# Autodesk Inventor assembly: Two stage cylindrical spur gear reducer with lateral offset
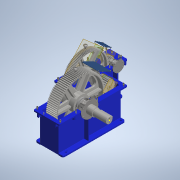
[picture p0: Inventor's stored thumbnail of the model, 180x180]
Saved by Autodesk Inventor 2020 (Build 240168000, 168)
## iProperties
Part Number: Two stage cylindrical spur gear reducer with lateral offset
Document SubType Name: 部件
Designer: chenpeizhi66
Author: PeiZhi Chen
## Documents named in this file (59)
- C:\Users\dell\Desktop\最终上交\爆炸图\装配3\Workspace\cpz assemble.iam
- C:\Users\dell\Desktop\最终上交\爆炸图\装配3\Libraries\Content Center Files\zh-CN\GB_T 283 (NUP)\滚动轴承 NUP NUP 208 E GB_T 283.ipt
- C:\Users\dell\Desktop\最终上交\爆炸图\装配3\Libraries\Content Center Files\zh-CN\GB_T 283 (NUP)\滚动轴承 NUP NUP 2313 E GB_T 283.ipt
- C:\Users\dell\Desktop\最终上交\爆炸图\装配3\Libraries\Content Center Files\zh-CN\GB_T 276-94\滚动轴承 61922 GB_T 276-94.ipt
- C:\Users\dell\Desktop\最终上交\爆炸图\装配3\Workspace\xia(1).ipt
- C:\Users\dell\Desktop\最终上交\爆炸图\装配3\Workspace\轴1.ipt
- C:\Users\dell\Desktop\最终上交\爆炸图\装配3\Workspace\轴2.ipt
- C:\Users\dell\Desktop\最终上交\爆炸图\装配3\Workspace\轴3.ipt
- C:\Users\dell\Desktop\最终上交\爆炸图\装配3\Workspace\挡油板2.ipt
- C:\Users\dell\Desktop\最终上交\爆炸图\装配3\Workspace\轴套1.ipt
- C:\Users\dell\Desktop\最终上交\爆炸图\装配3\Workspace\key1.ipt
- C:\Users\dell\Desktop\最终上交\爆炸图\装配3\Workspace\key2.ipt
- C:\Users\dell\Desktop\最终上交\爆炸图\装配3\Workspace\key3.ipt
- C:\Users\dell\Desktop\最终上交\爆炸图\装配3\Workspace\key5.ipt
- C:\Users\dell\Desktop\最终上交\爆炸图\装配3\Workspace\shaft_try_1\设计加速器\正齿轮11.ipt
- C:\Users\dell\Desktop\最终上交\爆炸图\装配3\Workspace\shaft_try_1\设计加速器\正齿轮12.ipt
- C:\Users\dell\Desktop\最终上交\爆炸图\装配3\Workspace\shaft_try_1\设计加速器\正齿轮21.ipt
- C:\Users\dell\Desktop\最终上交\爆炸图\装配3\Workspace\shaft_try_1\设计加速器\正齿轮22.ipt
- C:\Users\dell\Desktop\最终上交\爆炸图\装配3\Workspace\轴套3.ipt
- C:\Users\dell\Desktop\最终上交\爆炸图\装配3\Workspace\轴端挡圈.ipt
- C:\Users\dell\Desktop\最终上交\爆炸图\装配3\Workspace\螺栓 GB 32.1 M6 x 30.ipt
- C:\Users\dell\Desktop\最终上交\爆炸图\装配3\Workspace\轴套2.ipt
- C:\Users\dell\Desktop\最终上交\爆炸图\装配3\Workspace\弹性挡圈GB 894.1-86 - 40.ipt
- C:\Users\dell\Desktop\最终上交\爆炸图\装配3\Workspace\弹性挡圈GB 894.1-86 - 70.ipt
- C:\Users\dell\Desktop\最终上交\爆炸图\装配3\Workspace\轴4.ipt
- C:\Users\dell\Desktop\最终上交\爆炸图\装配3\Workspace\油塞1.ipt
- C:\Users\dell\Desktop\最终上交\爆炸图\装配3\Workspace\shang(1).ipt
- C:\Users\dell\Desktop\最终上交\爆炸图\装配3\Libraries\Content Center Files\zh-CN\GB_T 6175-2000\螺母 GB_T 6175 M10.ipt
- C:\Users\dell\Desktop\最终上交\爆炸图\装配3\Workspace\螺栓 GB_T 5785 M12 x 1.5 x 110.ipt
- C:\Users\dell\Desktop\最终上交\爆炸图\装配3\Workspace\螺栓 GB_T 5785 M12 x 1.5 x 45.ipt
- C:\Users\dell\Desktop\最终上交\爆炸图\装配3\Libraries\Content Center Files\zh-CN\GB 93-87\垫圈 GB 93-87 12.ipt
- C:\Users\dell\Desktop\最终上交\爆炸图\装配3\Workspace\螺母 GB_T 6175 M10.ipt
- C:\Users\dell\Desktop\最终上交\爆炸图\装配3\Workspace\视空盖1.ipt
- C:\Users\dell\Desktop\最终上交\爆炸图\装配3\Workspace\视孔盖2.ipt
- C:\Users\dell\Desktop\最终上交\爆炸图\装配3\Workspace\通气器1.ipt
- C:\Users\dell\Desktop\最终上交\爆炸图\装配3\Workspace\螺栓 GB_T 5783 M6 x 14.ipt
- C:\Users\dell\Desktop\最终上交\爆炸图\装配3\Libraries\Content Center Files\zh-CN\GB_T 5783-2000\螺栓 GB_T 5783 M6 x 14.ipt
- C:\Users\dell\Desktop\最终上交\爆炸图\装配3\Workspace\垫片1.ipt
- C:\Users\dell\Desktop\最终上交\爆炸图\装配3\Workspace\轴承端盖1.ipt
- C:\Users\dell\Desktop\最终上交\爆炸图\装配3\Workspace\O 形密封圈  P- 37.5 x 2.65-G-GB_T 3452.1-2005.ipt
- C:\Users\dell\Desktop\最终上交\爆炸图\装配3\Workspace\轴承端盖2.ipt
- C:\Users\dell\Desktop\最终上交\爆炸图\装配3\Workspace\垫片2.ipt
- C:\Users\dell\Desktop\最终上交\爆炸图\装配3\Workspace\垫片3.ipt
- C:\Users\dell\Desktop\最终上交\爆炸图\装配3\Workspace\垫片4.ipt
- C:\Users\dell\Desktop\最终上交\爆炸图\装配3\Workspace\轴承盖挡圈.ipt
- C:\Users\dell\Desktop\最终上交\爆炸图\装配3\Workspace\轴承通盖1.ipt
- C:\Users\dell\Desktop\最终上交\爆炸图\装配3\Workspace\轴承端盖3.ipt
- C:\Users\dell\Desktop\最终上交\爆炸图\装配3\Workspace\轴承通盖.ipt
- C:\Users\dell\Desktop\最终上交\爆炸图\装配3\Workspace\螺母 GB 810 M30 x 1.5.ipt
- C:\Users\dell\Desktop\最终上交\爆炸图\装配3\Libraries\Content Center Files\zh-CN\GB 858-88\垫圈 GB 858 30.ipt
- C:\Users\dell\Desktop\最终上交\爆炸图\装配3\Workspace\垫圈 GB 858 64.ipt
- C:\Users\dell\Desktop\最终上交\爆炸图\装配3\Workspace\螺母 GB 810 M64 x 2.ipt
- C:\Users\dell\Desktop\最终上交\爆炸图\装配3\Workspace\油塞垫.ipt
- C:\Users\dell\Desktop\最终上交\爆炸图\装配3\Workspace\锥形销 GB_T 117 A 10 x 40.ipt
- C:\Users\dell\Desktop\最终上交\爆炸图\装配3\Libraries\Content Center Files\zh-CN\GB_T 5782-2000\螺栓 GB_T 5782 M10 x 35.ipt
- C:\Users\dell\Desktop\最终上交\爆炸图\装配3\Workspace\零件2.ipt
- C:\Users\dell\Desktop\最终上交\爆炸图\装配3\Libraries\Content Center Files\zh-CN\GB 831-88\螺钉 GB 831 M8 x 6.ipt
- C:\Users\dell\Desktop\最终上交\爆炸图\装配3\Workspace\零件1.ipt
- C:\Users\dell\Desktop\最终上交\爆炸图\装配3\Workspace\零件3.ipt
## Components (146 placed, 54 different names)
1. 滚动轴承 GB/T 283 NUP 型 NUP 208 E:1 — 配合:2, 配合:18, 配合:54
2. 滚动轴承 GB/T 283 NUP 型 NUP 2313 E:1 — 配合:13, 配合:50, 配合:52
3. 滚动轴承 GB/T 283 NUP 型 NUP 208 E:2 — 配合:4, 配合:6, 配合:8, 配合:330, 配合:331, 配合:338
4. 滚动轴承 GB/T 283 NUP 型 NUP 2313 E:2 — 配合:14, 配合:15, 配合:16, 配合:334
5. 滚动轴承 GB/T 276-1994 60000 和 160000 型 61922:1 — 配合:23, 配合:29, 配合:419
6. 滚动轴承 GB/T 276-1994 60000 和 160000 型 61922:2 — 配合:24, 配合:38, 配合:418
7. xia(1):1 — 配合:2, 配合:4, 总驱动, 配合:5, 配合:11, 配合:12, 配合:13, 配合:14, 配合:15, 配合:23, 配合:24, 配合:59, 配合:60, 配合:65, 表面齐平:1, 表面齐平:2, 配合:66, 配合:67, 配合:68, 配合:69, 配合:70, 配合:71, 配合:72, 配合:73, 配合:74, 配合:75, 配合:76, 配合:77, 配合:78, 配合:79, 配合:80, 配合:81, 配合:82, 配合:83, 配合:84, 配合:85, 配合:108, 配合:109, 配合:110, 配合:111, 配合:112, 配合:113, 配合:114, 配合:115, 配合:116, 配合:117, 配合:118, 配合:119, 表面齐平:3, 表面齐平:4, 表面齐平:5, 表面齐平:6, 配合:298, 配合:307, 角度:2, 配合:318, 配合:319, 配合:320, 配合:322, 角度:3, 配合:327, 配合:340, 配合:341, 配合:342, 配合:344, 配合:345, 配合:346, 配合:362, 配合:364, 配合:366, 配合:368, 配合:370, 配合:372, 配合:374, 配合:376, 配合:388, 配合:390, 配合:392, 配合:400, 配合:402, 配合:404, 配合:416
8. shang(1):1 — 配合:65, 表面齐平:1, 表面齐平:2, 配合:163, 配合:165, 配合:167, 配合:169, 配合:171, 配合:173, 配合:175, 配合:177, 配合:179, 配合:181, 配合:183, 配合:185, 配合:187, 配合:189, 配合:191, 配合:193, 表面齐平:3, 表面齐平:4, 表面齐平:5, 表面齐平:6, 配合:269, 配合:270, 配合:271, 配合:272, 配合:273, 配合:274, 配合:275, 配合:276, 配合:277, 配合:278, 配合:279, 配合:281, 配合:283, 配合:285, 配合:287, 配合:289, 配合:291, 配合:293, 配合:299, 配合:308, 配合:312, 配合:314, 配合:315, 配合:349, 配合:350, 配合:352, 配合:354, 配合:356, 配合:358, 配合:360, 配合:378, 配合:380, 配合:382, 配合:384, 配合:386, 配合:394, 配合:396, 配合:398, 配合:407, 配合:408, 配合:409, 配合:410, 配合:411, 配合:412, 配合:413, 配合:414, 配合:415, 配合:417
9. 轴:1 — 配合:11, 刚性:3, 转动:1, 配合:16, 刚性:8, 配合:19, 配合:20, 转动:2, 配合:46, 配合:47, 配合:48, 配合:51, 配合:306, 配合:309, 配合:333, 配合:335, 刚性:10
10. 轴:2 — 配合:12, 转动:2, 配合:22, 配合:29, 配合:36, 配合:311, 配合:313, 配合:324, 配合:326, 刚性:11, 刚性:12
11. 驱动轴 — 总驱动, 配合:5, 配合:6, 配合:7, 配合:9, 刚性:1, 刚性:2, 配合:10, 转动:1, 配合:53, 配合:297, 配合:304, 配合:329, 配合:337
12. 挡油板2:1 — 配合:7, 配合:8, 配合:9
13. 轴套1:1 — 配合:10, 配合:17, 配合:18
14. key1:1 — 刚性:1
15. key2:1 — 刚性:2, 刚性:7
16. key3:1 — 刚性:3
17. key5:1 — 刚性:12, 配合:420
18. 正齿轮1:2 — 刚性:7, 配合:17
19. 正齿轮2:1 — 配合:22, 配合:37, 配合:420
20. 正齿轮2:2 — 刚性:8, 配合:49
21. 轴套3:1 — 配合:36, 配合:37, 配合:38
22. 轴端挡圈:1 — 配合:41, 配合:42, 配合:43, 配合:44, 配合:45, 对称:1
23. 螺栓 GB 32.1 M6 x 30:1 — 配合:43, 配合:45, 配合:47
24. 螺栓 GB 32.1 M6 x 30:2 — 配合:42, 配合:44, 配合:46, 对称:1, 表面齐平:9
25. 轴套2:1 — 配合:48, 配合:49, 配合:50
26. 弹性挡圈GB 894.1-86 - 40:1 — 配合:53, 配合:54
27. 弹性挡圈GB 894.1-86 - 70:1 — 配合:51, 配合:52
28. 轴:4 — 配合:59, 配合:60
29. 螺栓 GB_T 5785 M12 x 1.5 x 110:1 — 配合:66, 配合:67, 配合:132, 配合:164
30. 螺栓 GB_T 5785 M12 x 1.5 x 110:2 — 配合:68, 配合:69, 配合:178, 配合:208
31. 螺栓 GB_T 5785 M12 x 1.5 x 110:3 — 配合:70, 配合:71, 配合:136, 配合:168
32. 螺栓 GB_T 5785 M12 x 1.5 x 110:4 — 配合:72, 配合:73, 配合:186, 配合:216
33. 螺栓 GB_T 5785 M12 x 1.5 x 110:5 — 配合:74, 配合:75, 配合:134, 配合:166
34. 螺栓 GB_T 5785 M12 x 1.5 x 110:6 — 配合:76, 配合:77, 配合:106, 配合:162
35. 螺栓 GB_T 5785 M12 x 1.5 x 110:7 — 配合:78, 配合:79, 配合:184, 配合:214
36. 螺栓 GB_T 5785 M12 x 1.5 x 110:8 — 配合:80, 配合:81, 配合:188, 配合:218
37. 螺栓 GB_T 5785 M12 x 1.5 x 110:9 — 配合:82, 配合:83, 配合:180, 配合:210
38. 螺栓 GB_T 5785 M12 x 1.5 x 110:10 — 配合:84, 配合:85, 配合:172, 配合:202
39. 螺母 GB_T 6175 M10:1 — 配合:106, 配合:195
40. 螺栓 GB_T 5785 M12 x 1.5 x 45:1 — 配合:108, 配合:109, 配合:176, 配合:206
41. 螺栓 GB_T 5785 M12 x 1.5 x 45:2 — 配合:110, 配合:111, 配合:174, 配合:204
42. 螺栓 GB_T 5785 M12 x 1.5 x 45:3 — 配合:112, 配合:113, 配合:182, 配合:212
43. 螺栓 GB_T 5785 M12 x 1.5 x 45:4 — 配合:114, 配合:115, 配合:192, 配合:200
44. 螺栓 GB_T 5785 M12 x 1.5 x 45:5 — 配合:116, 配合:117, 配合:190, 配合:220
45. 螺栓 GB_T 5785 M12 x 1.5 x 45:6 — 配合:118, 配合:119, 配合:138, 配合:170
46. 螺母 GB_T 6175 M10:2 — 配合:132, 配合:196
47. 螺母 GB_T 6175 M10:3 — 配合:134, 配合:197
48. 螺母 GB_T 6175 M10:4 — 配合:136, 配合:198
49. 螺母 GB_T 6175 M10:5 — 配合:138, 配合:199
50. 垫圈 GB/T 93-1987 M12:1 — 配合:162, 配合:163, 配合:195
51. 垫圈 GB/T 93-1987 M12:2 — 配合:164, 配合:165, 配合:196
52. 垫圈 GB/T 93-1987 M12:3 — 配合:166, 配合:167, 配合:197
53. 垫圈 GB/T 93-1987 M12:4 — 配合:168, 配合:169, 配合:198
54. 垫圈 GB/T 93-1987 M12:5 — 配合:170, 配合:171, 配合:199
55. 垫圈 GB/T 93-1987 M12:6 — 配合:172, 配合:173, 配合:203
56. 垫圈 GB/T 93-1987 M12:7 — 配合:174, 配合:175, 配合:205
57. 垫圈 GB/T 93-1987 M12:8 — 配合:176, 配合:177, 配合:207
58. 垫圈 GB/T 93-1987 M12:9 — 配合:178, 配合:179, 配合:209
59. 垫圈 GB/T 93-1987 M12:10 — 配合:180, 配合:181, 配合:211
60. 垫圈 GB/T 93-1987 M12:11 — 配合:182, 配合:183, 配合:213
61. 垫圈 GB/T 93-1987 M12:12 — 配合:184, 配合:185, 配合:215
62. 垫圈 GB/T 93-1987 M12:13 — 配合:186, 配合:187, 配合:217
63. 垫圈 GB/T 93-1987 M12:14 — 配合:188, 配合:189, 配合:219
64. 垫圈 GB/T 93-1987 M12:15 — 配合:190, 配合:191, 配合:221
65. 垫圈 GB/T 93-1987 M12:16 — 配合:192, 配合:193, 配合:201
66. 螺母 GB/T 6175-2000 M10:1 — 配合:200, 配合:201
67. 螺母 GB/T 6175-2000 M10:2 — 配合:202, 配合:203
68. 螺母 GB/T 6175-2000 M10:3 — 配合:204, 配合:205
69. 螺母 GB/T 6175-2000 M10:4 — 配合:206, 配合:207
70. 螺母 GB/T 6175-2000 M10:5 — 配合:208, 配合:209
71. 螺母 GB/T 6175-2000 M10:6 — 配合:210, 配合:211
72. 螺母 GB/T 6175-2000 M10:7 — 配合:212, 配合:213
73. 螺母 GB/T 6175-2000 M10:8 — 配合:214, 配合:215
74. 螺母 GB/T 6175-2000 M10:9 — 配合:216, 配合:217
75. 螺母 GB/T 6175-2000 M10:10 — 配合:218, 配合:219
76. 螺母 GB/T 6175-2000 M10:11 — 配合:220, 配合:221
77. 视空盖1:1 — 配合:273, 配合:274, 配合:278, 配合:280, 配合:282, 配合:284, 配合:286
78. 视孔盖2:1 — 配合:275, 配合:276, 配合:277, 配合:288, 配合:290, 配合:292, 配合:294
79. 通气器1:1 — 配合:271, 配合:272
80. 通气器1:2 — 配合:269, 配合:270
81. 螺栓 GB_T 5783 M6 x 14:1 — 配合:279, 配合:280
82. 螺栓 GB_T 5783 M6 x 14:2 — 配合:281, 配合:282
83. 螺栓 GB_T 5783 M6 x 14:3 — 配合:283, 配合:284
84. 螺栓 GB_T 5783 M6 x 14:4 — 配合:285, 配合:286
85. 螺栓 GB/T 5783-2000 M6 x 14:1 — 配合:287, 配合:288
86. 螺栓 GB/T 5783-2000 M6 x 14:2 — 配合:289, 配合:290
87. 螺栓 GB/T 5783-2000 M6 x 14:3 — 配合:291, 配合:292
88. 螺栓 GB/T 5783-2000 M6 x 14:4 — 配合:293, 配合:294
89. 垫片1:1 — 配合:297, 配合:298, 配合:299, 配合:305
90. 轴承端盖1:1 — 配合:301, 配合:302, 配合:303, 配合:304, 配合:305, 配合:351, 配合:353, 配合:355, 配合:357, 配合:359, 配合:361, 配合:363, 配合:365, 配合:367, 配合:369, 配合:371, 配合:373
91. O 形密封圈  P- 37.5 x 2.65-G-GB_T 3452.1-2005:1 — 配合:301, 配合:302, 配合:303
92. 轴承端盖2:1 — 配合:309, 配合:310
93. 垫片2:1 — 配合:306, 配合:307, 配合:308, 配合:310
94. 垫片3:1 — 配合:311, 角度:2, 配合:312, 配合:325
95. 垫片4:1 — 配合:313, 配合:314, 配合:315, 配合:328
96. 垫片1:2 — 配合:318, 配合:319, 配合:320, 配合:323
97. 轴承通盖1:1 — 配合:322, 配合:323, 配合:395, 配合:397, 配合:399, 配合:401, 配合:403, 配合:405
98. 轴承端盖3:1 — 配合:324, 角度:3, 配合:325, 配合:375, 配合:377, 配合:379, 配合:381, 配合:419
99. 轴承通盖:1 — 配合:326, 配合:327, 配合:328, 配合:383, 配合:385, 配合:387, 配合:389, 配合:391, 配合:393, 配合:418, 表面齐平:7
100. 螺母 GB 810 M30 x 1.5:1 — 配合:331, 配合:332
101. 垫圈 GB/T 858-1988 30 x 40:1 — 配合:329, 配合:330, 配合:332
102. 垫圈 GB 858 64:1 — 配合:333, 配合:334, 配合:336
103. 螺母 GB 810 M64 x 2:1 — 配合:335, 配合:336
104. 轴承盖挡圈:2 — 配合:337, 配合:338
105. 油塞1:2 — 配合:342, 配合:343
106. 油塞垫:1 — 配合:344, 配合:345, 配合:347
107. 油塞垫:2 — 配合:340, 配合:341, 配合:343
108. 油塞1:3 — 配合:346, 配合:347
109. 锥形销 GB_T 117 A 10 x 40:1 — 配合:349, 配合:416
110. 螺栓 GB/T 5782-2000 M10x35:1 — 配合:350, 配合:351
111. 螺栓 GB/T 5782-2000 M10x35:2 — 配合:352, 配合:353
112. 螺栓 GB/T 5782-2000 M10x35:3 — 配合:354, 配合:355
113. 螺栓 GB/T 5782-2000 M10x35:4 — 配合:356, 配合:357
114. 螺栓 GB/T 5782-2000 M10x35:5 — 配合:358, 配合:359
115. 螺栓 GB/T 5782-2000 M10x35:6 — 配合:360, 配合:361
116. 螺栓 GB/T 5782-2000 M10x35:7 — 配合:362, 配合:363
117. 螺栓 GB/T 5782-2000 M10x35:8 — 配合:364, 配合:365
118. 螺栓 GB/T 5782-2000 M10x35:9 — 配合:366, 配合:367
119. 螺栓 GB/T 5782-2000 M10x35:10 — 配合:368, 配合:369
120. 螺栓 GB/T 5782-2000 M10x35:11 — 配合:370, 配合:371
121. 螺栓 GB/T 5782-2000 M10x35:12 — 配合:372, 配合:373
122. 螺栓 GB/T 5782-2000 M10x35:13 — 配合:374, 配合:375
123. 螺栓 GB/T 5782-2000 M10x35:14 — 配合:376, 配合:377
124. 螺栓 GB/T 5782-2000 M10x35:15 — 配合:378, 配合:379
125. 螺栓 GB/T 5782-2000 M10x35:16 — 配合:380, 配合:381
126. 螺栓 GB/T 5782-2000 M10x35:17 — 配合:382, 配合:383
127. 螺栓 GB/T 5782-2000 M10x35:18 — 配合:384, 配合:385
128. 螺栓 GB/T 5782-2000 M10x35:19 — 配合:386, 配合:387
129. 螺栓 GB/T 5782-2000 M10x35:20 — 配合:388, 配合:389
130. 螺栓 GB/T 5782-2000 M10x35:21 — 配合:390, 配合:391
131. 螺栓 GB/T 5782-2000 M10x35:22 — 配合:392, 配合:393
132. 螺栓 GB/T 5782-2000 M10x35:23 — 配合:394, 配合:395
133. 螺栓 GB/T 5782-2000 M10x35:24 — 配合:396, 配合:397
134. 螺栓 GB/T 5782-2000 M10x35:25 — 配合:398, 配合:399
135. 螺栓 GB/T 5782-2000 M10x35:26 — 配合:400, 配合:401
136. 螺栓 GB/T 5782-2000 M10x35:27 — 配合:402, 配合:403
137. 螺栓 GB/T 5782-2000 M10x35:28 — 配合:404, 配合:405
138. 零件2:1 — 刚性:10, 配合:406
139. 螺钉 GB/T 831-1988 M8 x 6:1 — 配合:407, 配合:408
140. 螺钉 GB/T 831-1988 M8 x 6:2 — 配合:409, 配合:417
141. 螺钉 GB/T 831-1988 M8 x 6:3 — 配合:410, 配合:414
142. 螺钉 GB/T 831-1988 M8 x 6:4 — 配合:411, 配合:413
143. 螺钉 GB/T 831-1988 M8 x 6:5 — 配合:412, 配合:415
144. 零件1:1 — 刚性:11
145. 零件3:1 — 表面齐平:7, 表面齐平:8, 表面齐平:9
146. 正齿轮1:1 — 配合:19, 配合:20, 配合:41, 配合:406
## Relationships (305: Mate 282, Flush 9, WeldJoint 8, Angle 3, RelateRotation 2, Symmetry 1)
- 配合:2 [Mate]: 滚动轴承 GB/T 283 NUP 型 NUP 208 E:1 ↔ xia(1):1
- 配合:4 [Mate]: 滚动轴承 GB/T 283 NUP 型 NUP 208 E:2 ↔ xia(1):1
- 总驱动 [Angle] (104 deg): xia(1):1 ↔ 驱动轴
- 配合:5 [Mate]: xia(1):1 ↔ 驱动轴
- 配合:6 [Mate]: 滚动轴承 GB/T 283 NUP 型 NUP 208 E:2 ↔ 驱动轴
- 配合:7 [Mate]: 驱动轴 ↔ 挡油板2:1
- 配合:8 [Mate]: 滚动轴承 GB/T 283 NUP 型 NUP 208 E:2 ↔ 挡油板2:1
- 配合:9 [Mate]: 驱动轴 ↔ 挡油板2:1
- 刚性:1 [WeldJoint]: 驱动轴 ↔ key1:1
- 刚性:2 [WeldJoint]: 驱动轴 ↔ key2:1
- 配合:10 [Mate]: 驱动轴 ↔ 轴套1:1
- 配合:11 [Mate]: xia(1):1 ↔ 轴:1
- 配合:12 [Mate]: xia(1):1 ↔ 轴:2
- 刚性:3 [WeldJoint]: 轴:1 ↔ key3:1
- 刚性:7 [WeldJoint]: key2:1 ↔ 正齿轮1:2
- 转动:1 [RelateRotation] (0.615 ul): 轴:1 ↔ 驱动轴
- 配合:13 [Mate]: 滚动轴承 GB/T 283 NUP 型 NUP 2313 E:1 ↔ xia(1):1
- 配合:14 [Mate]: 滚动轴承 GB/T 283 NUP 型 NUP 2313 E:2 ↔ xia(1):1
- 配合:15 [Mate]: 滚动轴承 GB/T 283 NUP 型 NUP 2313 E:2 ↔ xia(1):1
- 配合:16 [Mate]: 滚动轴承 GB/T 283 NUP 型 NUP 2313 E:2 ↔ 轴:1
- 配合:17 [Mate]: 轴套1:1 ↔ 正齿轮1:2
- 配合:18 [Mate]: 滚动轴承 GB/T 283 NUP 型 NUP 208 E:1 ↔ 轴套1:1
- 刚性:8 [WeldJoint]: 轴:1 ↔ 正齿轮2:2
- 配合:19 [Mate]: 轴:1 ↔ 正齿轮1:1
- 配合:20 [Mate]: 轴:1 ↔ 正齿轮1:1
- 转动:2 [RelateRotation] (1.833 ul): 轴:1 ↔ 轴:2
- 配合:22 [Mate]: 轴:2 ↔ 正齿轮2:1
- 配合:23 [Mate]: 滚动轴承 GB/T 276-1994 60000 和 160000 型 61922:1 ↔ xia(1):1
- 配合:24 [Mate]: 滚动轴承 GB/T 276-1994 60000 和 160000 型 61922:2 ↔ xia(1):1
- 配合:29 [Mate]: 滚动轴承 GB/T 276-1994 60000 和 160000 型 61922:1 ↔ 轴:2
- 配合:36 [Mate]: 轴:2 ↔ 轴套3:1
- 配合:37 [Mate]: 正齿轮2:1 ↔ 轴套3:1
- 配合:38 [Mate]: 滚动轴承 GB/T 276-1994 60000 和 160000 型 61922:2 ↔ 轴套3:1
- 配合:41 [Mate]: 轴端挡圈:1 ↔ 正齿轮1:1
- 配合:42 [Mate]: 轴端挡圈:1 ↔ 螺栓 GB 32.1 M6 x 30:2
- 配合:43 [Mate]: 轴端挡圈:1 ↔ 螺栓 GB 32.1 M6 x 30:1
- 配合:44 [Mate]: 轴端挡圈:1 ↔ 螺栓 GB 32.1 M6 x 30:2
- 配合:45 [Mate]: 轴端挡圈:1 ↔ 螺栓 GB 32.1 M6 x 30:1
- 配合:46 [Mate]: 轴:1 ↔ 螺栓 GB 32.1 M6 x 30:2
- 配合:47 [Mate]: 轴:1 ↔ 螺栓 GB 32.1 M6 x 30:1
- 配合:48 [Mate]: 轴:1 ↔ 轴套2:1
- 配合:49 [Mate]: 正齿轮2:2 ↔ 轴套2:1
- 配合:50 [Mate]: 滚动轴承 GB/T 283 NUP 型 NUP 2313 E:1 ↔ 轴套2:1
- 配合:51 [Mate]: 轴:1 ↔ 弹性挡圈GB 894.1-86 - 70:1
- 配合:52 [Mate]: 滚动轴承 GB/T 283 NUP 型 NUP 2313 E:1 ↔ 弹性挡圈GB 894.1-86 - 70:1
- 配合:53 [Mate]: 驱动轴 ↔ 弹性挡圈GB 894.1-86 - 40:1
- 配合:54 [Mate]: 滚动轴承 GB/T 283 NUP 型 NUP 208 E:1 ↔ 弹性挡圈GB 894.1-86 - 40:1
- 配合:59 [Mate]: xia(1):1 ↔ 轴:4
- 配合:60 [Mate]: xia(1):1 ↔ 轴:4
- 配合:65 [Mate]: xia(1):1 ↔ shang(1):1
- 表面齐平:1 [Flush]: xia(1):1 ↔ shang(1):1
- 表面齐平:2 [Flush]: xia(1):1 ↔ shang(1):1
- 配合:66 [Mate]: xia(1):1 ↔ 螺栓 GB_T 5785 M12 x 1.5 x 110:1
- 配合:67 [Mate]: xia(1):1 ↔ 螺栓 GB_T 5785 M12 x 1.5 x 110:1
- 配合:68 [Mate]: xia(1):1 ↔ 螺栓 GB_T 5785 M12 x 1.5 x 110:2
- 配合:69 [Mate]: xia(1):1 ↔ 螺栓 GB_T 5785 M12 x 1.5 x 110:2
- 配合:70 [Mate]: xia(1):1 ↔ 螺栓 GB_T 5785 M12 x 1.5 x 110:3
- 配合:71 [Mate]: xia(1):1 ↔ 螺栓 GB_T 5785 M12 x 1.5 x 110:3
- 配合:72 [Mate]: xia(1):1 ↔ 螺栓 GB_T 5785 M12 x 1.5 x 110:4
- 配合:73 [Mate]: xia(1):1 ↔ 螺栓 GB_T 5785 M12 x 1.5 x 110:4
- 配合:74 [Mate]: xia(1):1 ↔ 螺栓 GB_T 5785 M12 x 1.5 x 110:5
- 配合:75 [Mate]: xia(1):1 ↔ 螺栓 GB_T 5785 M12 x 1.5 x 110:5
- 配合:76 [Mate]: xia(1):1 ↔ 螺栓 GB_T 5785 M12 x 1.5 x 110:6
- 配合:77 [Mate]: xia(1):1 ↔ 螺栓 GB_T 5785 M12 x 1.5 x 110:6
- 配合:78 [Mate]: xia(1):1 ↔ 螺栓 GB_T 5785 M12 x 1.5 x 110:7
- 配合:79 [Mate]: xia(1):1 ↔ 螺栓 GB_T 5785 M12 x 1.5 x 110:7
- 配合:80 [Mate]: xia(1):1 ↔ 螺栓 GB_T 5785 M12 x 1.5 x 110:8
- 配合:81 [Mate]: xia(1):1 ↔ 螺栓 GB_T 5785 M12 x 1.5 x 110:8
- 配合:82 [Mate]: xia(1):1 ↔ 螺栓 GB_T 5785 M12 x 1.5 x 110:9
- 配合:83 [Mate]: xia(1):1 ↔ 螺栓 GB_T 5785 M12 x 1.5 x 110:9
- 配合:84 [Mate]: xia(1):1 ↔ 螺栓 GB_T 5785 M12 x 1.5 x 110:10
- 配合:85 [Mate]: xia(1):1 ↔ 螺栓 GB_T 5785 M12 x 1.5 x 110:10
- 配合:106 [Mate]: 螺栓 GB_T 5785 M12 x 1.5 x 110:6 ↔ 螺母 GB_T 6175 M10:1
- 配合:108 [Mate]: xia(1):1 ↔ 螺栓 GB_T 5785 M12 x 1.5 x 45:1
- 配合:109 [Mate]: xia(1):1 ↔ 螺栓 GB_T 5785 M12 x 1.5 x 45:1
- 配合:110 [Mate]: xia(1):1 ↔ 螺栓 GB_T 5785 M12 x 1.5 x 45:2
- 配合:111 [Mate]: xia(1):1 ↔ 螺栓 GB_T 5785 M12 x 1.5 x 45:2
- 配合:112 [Mate]: xia(1):1 ↔ 螺栓 GB_T 5785 M12 x 1.5 x 45:3
- 配合:113 [Mate]: xia(1):1 ↔ 螺栓 GB_T 5785 M12 x 1.5 x 45:3
- 配合:114 [Mate]: xia(1):1 ↔ 螺栓 GB_T 5785 M12 x 1.5 x 45:4
- 配合:115 [Mate]: xia(1):1 ↔ 螺栓 GB_T 5785 M12 x 1.5 x 45:4
- 配合:116 [Mate]: xia(1):1 ↔ 螺栓 GB_T 5785 M12 x 1.5 x 45:5
- 配合:117 [Mate]: xia(1):1 ↔ 螺栓 GB_T 5785 M12 x 1.5 x 45:5
- 配合:118 [Mate]: xia(1):1 ↔ 螺栓 GB_T 5785 M12 x 1.5 x 45:6
- 配合:119 [Mate]: xia(1):1 ↔ 螺栓 GB_T 5785 M12 x 1.5 x 45:6
- 配合:132 [Mate]: 螺栓 GB_T 5785 M12 x 1.5 x 110:1 ↔ 螺母 GB_T 6175 M10:2
- 配合:134 [Mate]: 螺栓 GB_T 5785 M12 x 1.5 x 110:5 ↔ 螺母 GB_T 6175 M10:3
- 配合:136 [Mate]: 螺栓 GB_T 5785 M12 x 1.5 x 110:3 ↔ 螺母 GB_T 6175 M10:4
- 配合:138 [Mate]: 螺栓 GB_T 5785 M12 x 1.5 x 45:6 ↔ 螺母 GB_T 6175 M10:5
- 配合:162 [Mate]: 螺栓 GB_T 5785 M12 x 1.5 x 110:6 ↔ 垫圈 GB/T 93-1987 M12:1
- 配合:163 [Mate]: shang(1):1 ↔ 垫圈 GB/T 93-1987 M12:1
- 配合:164 [Mate]: 螺栓 GB_T 5785 M12 x 1.5 x 110:1 ↔ 垫圈 GB/T 93-1987 M12:2
- 配合:165 [Mate]: shang(1):1 ↔ 垫圈 GB/T 93-1987 M12:2
- 配合:166 [Mate]: 螺栓 GB_T 5785 M12 x 1.5 x 110:5 ↔ 垫圈 GB/T 93-1987 M12:3
- 配合:167 [Mate]: shang(1):1 ↔ 垫圈 GB/T 93-1987 M12:3
- 配合:168 [Mate]: 螺栓 GB_T 5785 M12 x 1.5 x 110:3 ↔ 垫圈 GB/T 93-1987 M12:4
- 配合:169 [Mate]: shang(1):1 ↔ 垫圈 GB/T 93-1987 M12:4
- 配合:170 [Mate]: 螺栓 GB_T 5785 M12 x 1.5 x 45:6 ↔ 垫圈 GB/T 93-1987 M12:5
- 配合:171 [Mate]: shang(1):1 ↔ 垫圈 GB/T 93-1987 M12:5
- 配合:172 [Mate]: 螺栓 GB_T 5785 M12 x 1.5 x 110:10 ↔ 垫圈 GB/T 93-1987 M12:6
- 配合:173 [Mate]: shang(1):1 ↔ 垫圈 GB/T 93-1987 M12:6
- 配合:174 [Mate]: 螺栓 GB_T 5785 M12 x 1.5 x 45:2 ↔ 垫圈 GB/T 93-1987 M12:7
- 配合:175 [Mate]: shang(1):1 ↔ 垫圈 GB/T 93-1987 M12:7
- 配合:176 [Mate]: 螺栓 GB_T 5785 M12 x 1.5 x 45:1 ↔ 垫圈 GB/T 93-1987 M12:8
- 配合:177 [Mate]: shang(1):1 ↔ 垫圈 GB/T 93-1987 M12:8
- 配合:178 [Mate]: 螺栓 GB_T 5785 M12 x 1.5 x 110:2 ↔ 垫圈 GB/T 93-1987 M12:9
- 配合:179 [Mate]: shang(1):1 ↔ 垫圈 GB/T 93-1987 M12:9
- 配合:180 [Mate]: 螺栓 GB_T 5785 M12 x 1.5 x 110:9 ↔ 垫圈 GB/T 93-1987 M12:10
- 配合:181 [Mate]: shang(1):1 ↔ 垫圈 GB/T 93-1987 M12:10
- 配合:182 [Mate]: 螺栓 GB_T 5785 M12 x 1.5 x 45:3 ↔ 垫圈 GB/T 93-1987 M12:11
- 配合:183 [Mate]: shang(1):1 ↔ 垫圈 GB/T 93-1987 M12:11
- 配合:184 [Mate]: 螺栓 GB_T 5785 M12 x 1.5 x 110:7 ↔ 垫圈 GB/T 93-1987 M12:12
- 配合:185 [Mate]: shang(1):1 ↔ 垫圈 GB/T 93-1987 M12:12
- 配合:186 [Mate]: 螺栓 GB_T 5785 M12 x 1.5 x 110:4 ↔ 垫圈 GB/T 93-1987 M12:13
- 配合:187 [Mate]: shang(1):1 ↔ 垫圈 GB/T 93-1987 M12:13
- 配合:188 [Mate]: 螺栓 GB_T 5785 M12 x 1.5 x 110:8 ↔ 垫圈 GB/T 93-1987 M12:14
- 配合:189 [Mate]: shang(1):1 ↔ 垫圈 GB/T 93-1987 M12:14
- 配合:190 [Mate]: 螺栓 GB_T 5785 M12 x 1.5 x 45:5 ↔ 垫圈 GB/T 93-1987 M12:15
- 配合:191 [Mate]: shang(1):1 ↔ 垫圈 GB/T 93-1987 M12:15
- 配合:192 [Mate]: 螺栓 GB_T 5785 M12 x 1.5 x 45:4 ↔ 垫圈 GB/T 93-1987 M12:16
- 配合:193 [Mate]: shang(1):1 ↔ 垫圈 GB/T 93-1987 M12:16
- 配合:195 [Mate]: 螺母 GB_T 6175 M10:1 ↔ 垫圈 GB/T 93-1987 M12:1
- 配合:196 [Mate]: 螺母 GB_T 6175 M10:2 ↔ 垫圈 GB/T 93-1987 M12:2
- 配合:197 [Mate]: 螺母 GB_T 6175 M10:3 ↔ 垫圈 GB/T 93-1987 M12:3
- 配合:198 [Mate]: 螺母 GB_T 6175 M10:4 ↔ 垫圈 GB/T 93-1987 M12:4
- 配合:199 [Mate]: 螺母 GB_T 6175 M10:5 ↔ 垫圈 GB/T 93-1987 M12:5
- 配合:200 [Mate]: 螺栓 GB_T 5785 M12 x 1.5 x 45:4 ↔ 螺母 GB/T 6175-2000 M10:1
- 配合:201 [Mate]: 垫圈 GB/T 93-1987 M12:16 ↔ 螺母 GB/T 6175-2000 M10:1
- 配合:202 [Mate]: 螺栓 GB_T 5785 M12 x 1.5 x 110:10 ↔ 螺母 GB/T 6175-2000 M10:2
- 配合:203 [Mate]: 垫圈 GB/T 93-1987 M12:6 ↔ 螺母 GB/T 6175-2000 M10:2
- 配合:204 [Mate]: 螺栓 GB_T 5785 M12 x 1.5 x 45:2 ↔ 螺母 GB/T 6175-2000 M10:3
- 配合:205 [Mate]: 垫圈 GB/T 93-1987 M12:7 ↔ 螺母 GB/T 6175-2000 M10:3
- 配合:206 [Mate]: 螺栓 GB_T 5785 M12 x 1.5 x 45:1 ↔ 螺母 GB/T 6175-2000 M10:4
- 配合:207 [Mate]: 垫圈 GB/T 93-1987 M12:8 ↔ 螺母 GB/T 6175-2000 M10:4
- 配合:208 [Mate]: 螺栓 GB_T 5785 M12 x 1.5 x 110:2 ↔ 螺母 GB/T 6175-2000 M10:5
- 配合:209 [Mate]: 垫圈 GB/T 93-1987 M12:9 ↔ 螺母 GB/T 6175-2000 M10:5
- 配合:210 [Mate]: 螺栓 GB_T 5785 M12 x 1.5 x 110:9 ↔ 螺母 GB/T 6175-2000 M10:6
- 配合:211 [Mate]: 垫圈 GB/T 93-1987 M12:10 ↔ 螺母 GB/T 6175-2000 M10:6
- 配合:212 [Mate]: 螺栓 GB_T 5785 M12 x 1.5 x 45:3 ↔ 螺母 GB/T 6175-2000 M10:7
- 配合:213 [Mate]: 垫圈 GB/T 93-1987 M12:11 ↔ 螺母 GB/T 6175-2000 M10:7
- 配合:214 [Mate]: 螺栓 GB_T 5785 M12 x 1.5 x 110:7 ↔ 螺母 GB/T 6175-2000 M10:8
- 配合:215 [Mate]: 垫圈 GB/T 93-1987 M12:12 ↔ 螺母 GB/T 6175-2000 M10:8
- 配合:216 [Mate]: 螺栓 GB_T 5785 M12 x 1.5 x 110:4 ↔ 螺母 GB/T 6175-2000 M10:9
- 配合:217 [Mate]: 垫圈 GB/T 93-1987 M12:13 ↔ 螺母 GB/T 6175-2000 M10:9
- 配合:218 [Mate]: 螺栓 GB_T 5785 M12 x 1.5 x 110:8 ↔ 螺母 GB/T 6175-2000 M10:10
- 配合:219 [Mate]: 垫圈 GB/T 93-1987 M12:14 ↔ 螺母 GB/T 6175-2000 M10:10
- 配合:220 [Mate]: 螺栓 GB_T 5785 M12 x 1.5 x 45:5 ↔ 螺母 GB/T 6175-2000 M10:11
- 配合:221 [Mate]: 垫圈 GB/T 93-1987 M12:15 ↔ 螺母 GB/T 6175-2000 M10:11
- 表面齐平:3 [Flush]: xia(1):1 ↔ shang(1):1
- 表面齐平:4 [Flush]: xia(1):1 ↔ shang(1):1
- 表面齐平:5 [Flush]: xia(1):1 ↔ shang(1):1
- 表面齐平:6 [Flush]: xia(1):1 ↔ shang(1):1
- 配合:269 [Mate]: shang(1):1 ↔ 通气器1:2
- 配合:270 [Mate]: shang(1):1 ↔ 通气器1:2
- 配合:271 [Mate]: shang(1):1 ↔ 通气器1:1
- 配合:272 [Mate]: shang(1):1 ↔ 通气器1:1
- 配合:273 [Mate]: shang(1):1 ↔ 视空盖1:1
- 配合:274 [Mate]: shang(1):1 ↔ 视空盖1:1
- 配合:275 [Mate]: shang(1):1 ↔ 视孔盖2:1
- 配合:276 [Mate]: shang(1):1 ↔ 视孔盖2:1
- 配合:277 [Mate]: shang(1):1 ↔ 视孔盖2:1
- 配合:278 [Mate]: shang(1):1 ↔ 视空盖1:1
- 配合:279 [Mate]: shang(1):1 ↔ 螺栓 GB_T 5783 M6 x 14:1
- 配合:280 [Mate]: 视空盖1:1 ↔ 螺栓 GB_T 5783 M6 x 14:1
- 配合:281 [Mate]: shang(1):1 ↔ 螺栓 GB_T 5783 M6 x 14:2
- 配合:282 [Mate]: 视空盖1:1 ↔ 螺栓 GB_T 5783 M6 x 14:2
- 配合:283 [Mate]: shang(1):1 ↔ 螺栓 GB_T 5783 M6 x 14:3
- 配合:284 [Mate]: 视空盖1:1 ↔ 螺栓 GB_T 5783 M6 x 14:3
- 配合:285 [Mate]: shang(1):1 ↔ 螺栓 GB_T 5783 M6 x 14:4
- 配合:286 [Mate]: 视空盖1:1 ↔ 螺栓 GB_T 5783 M6 x 14:4
- 配合:287 [Mate]: shang(1):1 ↔ 螺栓 GB/T 5783-2000 M6 x 14:1
- 配合:288 [Mate]: 视孔盖2:1 ↔ 螺栓 GB/T 5783-2000 M6 x 14:1
- 配合:289 [Mate]: shang(1):1 ↔ 螺栓 GB/T 5783-2000 M6 x 14:2
- 配合:290 [Mate]: 视孔盖2:1 ↔ 螺栓 GB/T 5783-2000 M6 x 14:2
- 配合:291 [Mate]: shang(1):1 ↔ 螺栓 GB/T 5783-2000 M6 x 14:3
- 配合:292 [Mate]: 视孔盖2:1 ↔ 螺栓 GB/T 5783-2000 M6 x 14:3
- 配合:293 [Mate]: shang(1):1 ↔ 螺栓 GB/T 5783-2000 M6 x 14:4
- 配合:294 [Mate]: 视孔盖2:1 ↔ 螺栓 GB/T 5783-2000 M6 x 14:4
- 配合:297 [Mate]: 驱动轴 ↔ 垫片1:1
- 配合:298 [Mate]: xia(1):1 ↔ 垫片1:1
- 配合:299 [Mate]: shang(1):1 ↔ 垫片1:1
- 配合:301 [Mate]: 轴承端盖1:1 ↔ O 形密封圈  P- 37.5 x 2.65-G-GB_T 3452.1-2005:1
- 配合:302 [Mate]: 轴承端盖1:1 ↔ O 形密封圈  P- 37.5 x 2.65-G-GB_T 3452.1-2005:1
- 配合:303 [Mate]: 轴承端盖1:1 ↔ O 形密封圈  P- 37.5 x 2.65-G-GB_T 3452.1-2005:1
- 配合:304 [Mate]: 驱动轴 ↔ 轴承端盖1:1
- 配合:305 [Mate]: 垫片1:1 ↔ 轴承端盖1:1
- 配合:306 [Mate]: 轴:1 ↔ 垫片2:1
- 配合:307 [Mate]: xia(1):1 ↔ 垫片2:1
- 配合:308 [Mate]: shang(1):1 ↔ 垫片2:1
- 配合:309 [Mate]: 轴:1 ↔ 轴承端盖2:1
- 配合:310 [Mate]: 轴承端盖2:1 ↔ 垫片2:1
- 配合:311 [Mate]: 轴:2 ↔ 垫片3:1
- 角度:2 [Angle] (180 deg): xia(1):1 ↔ 垫片3:1
- 配合:312 [Mate]: shang(1):1 ↔ 垫片3:1
- 配合:313 [Mate]: 轴:2 ↔ 垫片4:1
- 配合:314 [Mate]: shang(1):1 ↔ 垫片4:1
- 配合:315 [Mate]: shang(1):1 ↔ 垫片4:1
- 配合:318 [Mate]: xia(1):1 ↔ 垫片1:2
- 配合:319 [Mate]: xia(1):1 ↔ 垫片1:2
- 配合:320 [Mate]: xia(1):1 ↔ 垫片1:2
- 配合:322 [Mate]: xia(1):1 ↔ 轴承通盖1:1
- 配合:323 [Mate]: 垫片1:2 ↔ 轴承通盖1:1
- 配合:324 [Mate]: 轴:2 ↔ 轴承端盖3:1
- 角度:3 [Angle] (180 deg): xia(1):1 ↔ 轴承端盖3:1
- 配合:325 [Mate]: 垫片3:1 ↔ 轴承端盖3:1
- 配合:326 [Mate]: 轴:2 ↔ 轴承通盖:1
- 配合:327 [Mate]: xia(1):1 ↔ 轴承通盖:1
- 配合:328 [Mate]: 垫片4:1 ↔ 轴承通盖:1
- 配合:329 [Mate]: 驱动轴 ↔ 垫圈 GB/T 858-1988 30 x 40:1
- 配合:330 [Mate]: 滚动轴承 GB/T 283 NUP 型 NUP 208 E:2 ↔ 垫圈 GB/T 858-1988 30 x 40:1
- 配合:331 [Mate]: 滚动轴承 GB/T 283 NUP 型 NUP 208 E:2 ↔ 螺母 GB 810 M30 x 1.5:1
- 配合:332 [Mate]: 螺母 GB 810 M30 x 1.5:1 ↔ 垫圈 GB/T 858-1988 30 x 40:1
- 配合:333 [Mate]: 轴:1 ↔ 垫圈 GB 858 64:1
- 配合:334 [Mate]: 滚动轴承 GB/T 283 NUP 型 NUP 2313 E:2 ↔ 垫圈 GB 858 64:1
- 配合:335 [Mate]: 轴:1 ↔ 螺母 GB 810 M64 x 2:1
- 配合:336 [Mate]: 垫圈 GB 858 64:1 ↔ 螺母 GB 810 M64 x 2:1
- 配合:337 [Mate]: 驱动轴 ↔ 轴承盖挡圈:2
- 配合:338 [Mate]: 滚动轴承 GB/T 283 NUP 型 NUP 208 E:2 ↔ 轴承盖挡圈:2
- 配合:340 [Mate]: xia(1):1 ↔ 油塞垫:2
- 配合:341 [Mate]: xia(1):1 ↔ 油塞垫:2
- 配合:342 [Mate]: xia(1):1 ↔ 油塞1:2
- 配合:343 [Mate]: 油塞1:2 ↔ 油塞垫:2
- 配合:344 [Mate]: xia(1):1 ↔ 油塞垫:1
- 配合:345 [Mate]: xia(1):1 ↔ 油塞垫:1
- 配合:346 [Mate]: xia(1):1 ↔ 油塞1:3
- 配合:347 [Mate]: 油塞垫:1 ↔ 油塞1:3
- 配合:349 [Mate] (-9 mm): shang(1):1 ↔ 锥形销 GB_T 117 A 10 x 40:1
- 配合:350 [Mate]: shang(1):1 ↔ 螺栓 GB/T 5782-2000 M10x35:1
- 配合:351 [Mate]: 轴承端盖1:1 ↔ 螺栓 GB/T 5782-2000 M10x35:1
- 配合:352 [Mate]: shang(1):1 ↔ 螺栓 GB/T 5782-2000 M10x35:2
- 配合:353 [Mate]: 轴承端盖1:1 ↔ 螺栓 GB/T 5782-2000 M10x35:2
- 配合:354 [Mate]: shang(1):1 ↔ 螺栓 GB/T 5782-2000 M10x35:3
- 配合:355 [Mate]: 轴承端盖1:1 ↔ 螺栓 GB/T 5782-2000 M10x35:3
- 配合:356 [Mate]: shang(1):1 ↔ 螺栓 GB/T 5782-2000 M10x35:4
- 配合:357 [Mate]: 轴承端盖1:1 ↔ 螺栓 GB/T 5782-2000 M10x35:4
- 配合:358 [Mate]: shang(1):1 ↔ 螺栓 GB/T 5782-2000 M10x35:5
- 配合:359 [Mate]: 轴承端盖1:1 ↔ 螺栓 GB/T 5782-2000 M10x35:5
- 配合:360 [Mate]: shang(1):1 ↔ 螺栓 GB/T 5782-2000 M10x35:6
- 配合:361 [Mate]: 轴承端盖1:1 ↔ 螺栓 GB/T 5782-2000 M10x35:6
- 配合:362 [Mate]: xia(1):1 ↔ 螺栓 GB/T 5782-2000 M10x35:7
- 配合:363 [Mate]: 轴承端盖1:1 ↔ 螺栓 GB/T 5782-2000 M10x35:7
- 配合:364 [Mate]: xia(1):1 ↔ 螺栓 GB/T 5782-2000 M10x35:8
- 配合:365 [Mate]: 轴承端盖1:1 ↔ 螺栓 GB/T 5782-2000 M10x35:8
- 配合:366 [Mate]: xia(1):1 ↔ 螺栓 GB/T 5782-2000 M10x35:9
- 配合:367 [Mate]: 轴承端盖1:1 ↔ 螺栓 GB/T 5782-2000 M10x35:9
- 配合:368 [Mate]: xia(1):1 ↔ 螺栓 GB/T 5782-2000 M10x35:10
- 配合:369 [Mate]: 轴承端盖1:1 ↔ 螺栓 GB/T 5782-2000 M10x35:10
- 配合:370 [Mate]: xia(1):1 ↔ 螺栓 GB/T 5782-2000 M10x35:11
- 配合:371 [Mate]: 轴承端盖1:1 ↔ 螺栓 GB/T 5782-2000 M10x35:11
- 配合:372 [Mate]: xia(1):1 ↔ 螺栓 GB/T 5782-2000 M10x35:12
- 配合:373 [Mate]: 轴承端盖1:1 ↔ 螺栓 GB/T 5782-2000 M10x35:12
- 配合:374 [Mate]: xia(1):1 ↔ 螺栓 GB/T 5782-2000 M10x35:13
- 配合:375 [Mate]: 轴承端盖3:1 ↔ 螺栓 GB/T 5782-2000 M10x35:13
- 配合:376 [Mate]: xia(1):1 ↔ 螺栓 GB/T 5782-2000 M10x35:14
- 配合:377 [Mate]: 轴承端盖3:1 ↔ 螺栓 GB/T 5782-2000 M10x35:14
- 配合:378 [Mate]: shang(1):1 ↔ 螺栓 GB/T 5782-2000 M10x35:15
- 配合:379 [Mate]: 轴承端盖3:1 ↔ 螺栓 GB/T 5782-2000 M10x35:15
- 配合:380 [Mate]: shang(1):1 ↔ 螺栓 GB/T 5782-2000 M10x35:16
- 配合:381 [Mate]: 轴承端盖3:1 ↔ 螺栓 GB/T 5782-2000 M10x35:16
- 配合:382 [Mate]: shang(1):1 ↔ 螺栓 GB/T 5782-2000 M10x35:17
- 配合:383 [Mate]: 轴承通盖:1 ↔ 螺栓 GB/T 5782-2000 M10x35:17
- 配合:384 [Mate]: shang(1):1 ↔ 螺栓 GB/T 5782-2000 M10x35:18
- 配合:385 [Mate]: 轴承通盖:1 ↔ 螺栓 GB/T 5782-2000 M10x35:18
- 配合:386 [Mate]: shang(1):1 ↔ 螺栓 GB/T 5782-2000 M10x35:19
- 配合:387 [Mate]: 轴承通盖:1 ↔ 螺栓 GB/T 5782-2000 M10x35:19
- 配合:388 [Mate]: xia(1):1 ↔ 螺栓 GB/T 5782-2000 M10x35:20
- 配合:389 [Mate]: 轴承通盖:1 ↔ 螺栓 GB/T 5782-2000 M10x35:20
- 配合:390 [Mate]: xia(1):1 ↔ 螺栓 GB/T 5782-2000 M10x35:21
- 配合:391 [Mate]: 轴承通盖:1 ↔ 螺栓 GB/T 5782-2000 M10x35:21
- 配合:392 [Mate]: xia(1):1 ↔ 螺栓 GB/T 5782-2000 M10x35:22
- 配合:393 [Mate]: 轴承通盖:1 ↔ 螺栓 GB/T 5782-2000 M10x35:22
- 配合:394 [Mate]: shang(1):1 ↔ 螺栓 GB/T 5782-2000 M10x35:23
- 配合:395 [Mate]: 轴承通盖1:1 ↔ 螺栓 GB/T 5782-2000 M10x35:23
- 配合:396 [Mate]: shang(1):1 ↔ 螺栓 GB/T 5782-2000 M10x35:24
- 配合:397 [Mate]: 轴承通盖1:1 ↔ 螺栓 GB/T 5782-2000 M10x35:24
- 配合:398 [Mate]: shang(1):1 ↔ 螺栓 GB/T 5782-2000 M10x35:25
- 配合:399 [Mate]: 轴承通盖1:1 ↔ 螺栓 GB/T 5782-2000 M10x35:25
- 配合:400 [Mate]: xia(1):1 ↔ 螺栓 GB/T 5782-2000 M10x35:26
- 配合:401 [Mate]: 轴承通盖1:1 ↔ 螺栓 GB/T 5782-2000 M10x35:26
- 配合:402 [Mate]: xia(1):1 ↔ 螺栓 GB/T 5782-2000 M10x35:27
- 配合:403 [Mate]: 轴承通盖1:1 ↔ 螺栓 GB/T 5782-2000 M10x35:27
- 配合:404 [Mate]: xia(1):1 ↔ 螺栓 GB/T 5782-2000 M10x35:28
- 配合:405 [Mate]: 轴承通盖1:1 ↔ 螺栓 GB/T 5782-2000 M10x35:28
- 刚性:10 [WeldJoint]: 轴:1 ↔ 零件2:1
- 配合:406 [Mate]: 零件2:1 ↔ 正齿轮1:1
- 配合:407 [Mate]: shang(1):1 ↔ 螺钉 GB/T 831-1988 M8 x 6:1
- 配合:408 [Mate] (0.5 mm): shang(1):1 ↔ 螺钉 GB/T 831-1988 M8 x 6:1
- 配合:409 [Mate]: shang(1):1 ↔ 螺钉 GB/T 831-1988 M8 x 6:2
- 配合:410 [Mate]: shang(1):1 ↔ 螺钉 GB/T 831-1988 M8 x 6:3
- 配合:411 [Mate]: shang(1):1 ↔ 螺钉 GB/T 831-1988 M8 x 6:4
- 配合:412 [Mate]: shang(1):1 ↔ 螺钉 GB/T 831-1988 M8 x 6:5
- 配合:413 [Mate]: shang(1):1 ↔ 螺钉 GB/T 831-1988 M8 x 6:4
- 配合:414 [Mate]: shang(1):1 ↔ 螺钉 GB/T 831-1988 M8 x 6:3
- 配合:415 [Mate]: shang(1):1 ↔ 螺钉 GB/T 831-1988 M8 x 6:5
- 配合:416 [Mate]: xia(1):1 ↔ 锥形销 GB_T 117 A 10 x 40:1
- 配合:417 [Mate]: shang(1):1 ↔ 螺钉 GB/T 831-1988 M8 x 6:2
- 刚性:11 [WeldJoint]: 轴:2 ↔ 零件1:1
- 配合:418 [Mate]: 滚动轴承 GB/T 276-1994 60000 和 160000 型 61922:2 ↔ 轴承通盖:1
- 刚性:12 [WeldJoint]: 轴:2 ↔ key5:1
- 配合:419 [Mate]: 滚动轴承 GB/T 276-1994 60000 和 160000 型 61922:1 ↔ 轴承端盖3:1
- 配合:420 [Mate]: key5:1 ↔ 正齿轮2:1
- 表面齐平:7 [Flush]: 轴承通盖:1 ↔ 零件3:1
- 对称:1 [Symmetry]: 轴端挡圈:1 ↔ 螺栓 GB 32.1 M6 x 30:2
- 表面齐平:8 [Flush]: 零件3:1
- 表面齐平:9 [Flush]: 螺栓 GB 32.1 M6 x 30:2 ↔ 零件3:1
